# Autodesk Inventor assembly: Porsche_912_Standard_CV_Axle_Assembly
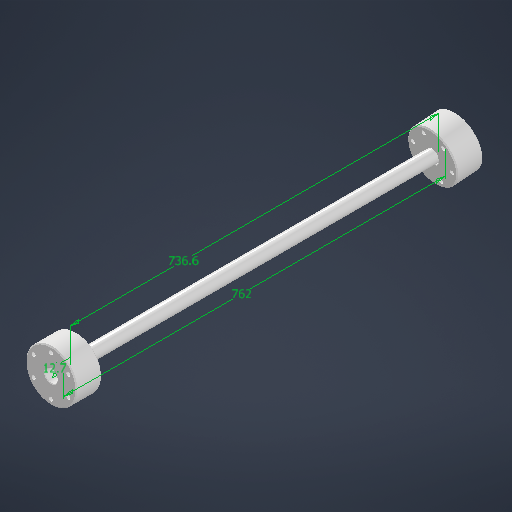
[picture p0: Inventor's stored thumbnail of the model, 512x512]
Saved by Autodesk Inventor 2026.1 (Build 301233000, 233)
## iProperties
Created: 2026-08-06
Part Number: Porsche_912_Standard_CV_Axle_Assembly
Document SubType Name: Assembly
Designer: share
Author: share
## Documents named in this file (3)
- C:\Users\share\OneDrive\Documents\Personal Projects\GOGO Kart\CAD\GOGO_KART_FSAE\Drivetrain\CV Axles\Porsche_912_Standard_CV_Axle_Assembly.iam
- C:\Users\share\OneDrive\Documents\Personal Projects\GOGO Kart\CAD\GOGO_KART_FSAE\Drivetrain\CV Axles\Porsche_912_CV_Joint.ipt
- C:\Users\share\OneDrive\Documents\Personal Projects\GOGO Kart\CAD\GOGO_KART_FSAE\Drivetrain\CV Axles\Porsche_912_Main_CV_Shaft.ipt
## Components (3 placed, 2 different names)
1. Porsche_912_CV_Joint:1 — Mate:2
2. Porsche_912_Main_CV_Shaft:1 — Mate:1, Mate:2, Flush:1, Flush:2, Flush:3
3. Porsche_912_CV_Joint:2 — Mate:1
## Relationships (5: Flush 3, Mate 2)
- Mate:1: Porsche_912_Main_CV_Shaft:1 ↔ Porsche_912_CV_Joint:2
- Mate:2: Porsche_912_CV_Joint:1 ↔ Porsche_912_Main_CV_Shaft:1
- Flush:1: Porsche_912_Main_CV_Shaft:1
- Flush:2: Porsche_912_Main_CV_Shaft:1
- Flush:3: Porsche_912_Main_CV_Shaft:1
